# Autodesk Inventor assembly: TestRig
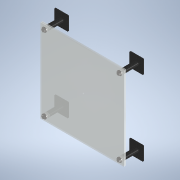
[picture p0: Inventor's stored thumbnail of the model, 180x180]
Saved by Autodesk Inventor 2020.3 (Build 243373010, 373A)
## iProperties
Created: 2020-10-30
Part Number: TestRig
Document SubType Name: Assembly
Designer: Naude Conradie
Author: Naude Conradie
## Documents named in this file (7)
- C:\Users\Naude Conradie\Desktop\Repository\Masters-Project\Models\Inventor\Testing Rig\TestRig.iam
- C:\Users\Naude Conradie\Desktop\Repository\Masters-Project\Models\Inventor\Testing Rig\Plate.ipt
- C:\Users\Naude Conradie\Desktop\Repository\Masters-Project\Models\Inventor\Testing Rig\PlateHoled.ipt
- C:\Users\Naude Conradie\Desktop\Repository\Masters-Project\Models\Inventor\Testing Rig\Leg.ipt
- C:\Users\Naude Conradie\Documents\Inventor\Content Center Files\R2020\en-US\ANSI B18.2.3.5M\ANSI B18.2.3.5M - M6 x 1 x 30.ipt
- C:\Users\Naude Conradie\Desktop\Repository\Masters-Project\Models\Inventor\Testing Rig\Washer.ipt
- C:\Users\Naude Conradie\Documents\Inventor\Content Center Files\R2020\en-US\IFI (3)\IFI - 6(9).ipt
## Components (22 placed, 6 different names)
1. Plate:1 — Mate:4, Flush:3, Mate:22, Mate:23, Mate:24, Mate:25, Mate:26, Mate:27, Mate:28, Mate:29, Mate:37, Mate:38, Mate:39, Mate:40, Mate:44, Mate:45, Mate:46, Mate:47, Angle:5, Angle:6, Angle:7, Angle:8
2. PlateHoled:1 — Mate:4, Flush:3, Mate:18, Mate:19, Mate:20, Mate:21, Angle:1, Angle:2, Angle:3, Angle:4, Mate:30, Mate:33, Mate:48, Mate:49, Mate:50
3. Leg:1 — Mate:18, Angle:1, Mate:35, Mate:43
4. Leg:2 — Mate:19, Angle:2, Mate:31, Mate:32
5. Leg:3 — Mate:20, Angle:3, Mate:34, Mate:42
6. Leg:4 — Mate:21, Angle:4, Mate:36, Mate:41
7. Hex Bolt - Metric M6 x 1 x 30:1 — Mate:51, Mate:57, Angle:7
8. Hex Bolt - Metric M6 x 1 x 30:2 — Mate:52, Mate:58, Angle:8
9. Hex Bolt - Metric M6 x 1 x 30:3 — Mate:53, Mate:55, Angle:5
10. Hex Bolt - Metric M6 x 1 x 30:4 — Mate:54, Mate:56, Angle:6
11. Washer:1 — Mate:22, Mate:27
12. Washer:2 — Mate:23, Mate:28
13. Washer:3 — Mate:25, Mate:29, Mate:30
14. Washer:4 — Mate:24, Mate:26
15. Round Test Washer (Metric) (IFI) 6:1 — Mate:31, Mate:32, Mate:33
16. Round Test Washer (Metric) (IFI) 6:2 — Mate:38, Mate:46, Mate:52, Mate:58
17. Round Test Washer (Metric) (IFI) 6:3 — Mate:39, Mate:45, Mate:51, Mate:57
18. Round Test Washer (Metric) (IFI) 6:4 — Mate:37, Mate:44, Mate:53, Mate:55
19. Round Test Washer (Metric) (IFI) 6:5 — Mate:40, Mate:47, Mate:54, Mate:56
20. Round Test Washer (Metric) (IFI) 6:6 — Mate:36, Mate:41, Mate:48
21. Round Test Washer (Metric) (IFI) 6:7 — Mate:35, Mate:43, Mate:50
22. Round Test Washer (Metric) (IFI) 6:8 — Mate:34, Mate:42, Mate:49
## Relationships (51: Mate 42, Angle 8, Flush 1)
- Mate:4: Plate:1 ↔ PlateHoled:1
- Flush:3: Plate:1 ↔ PlateHoled:1
- Mate:18: PlateHoled:1 ↔ Leg:1
- Mate:19: PlateHoled:1 ↔ Leg:2
- Mate:20: PlateHoled:1 ↔ Leg:3
- Mate:21: PlateHoled:1 ↔ Leg:4
- Angle:1 (0 deg): PlateHoled:1 ↔ Leg:1
- Angle:2 (0 deg): PlateHoled:1 ↔ Leg:2
- Angle:3 (0 deg): PlateHoled:1 ↔ Leg:3
- Angle:4 (0 deg): PlateHoled:1 ↔ Leg:4
- Mate:22: Plate:1 ↔ Washer:1
- Mate:23: Plate:1 ↔ Washer:2
- Mate:24: Plate:1 ↔ Washer:4
- Mate:25: Plate:1 ↔ Washer:3
- Mate:26: Plate:1 ↔ Washer:4
- Mate:27: Plate:1 ↔ Washer:1
- Mate:28: Plate:1 ↔ Washer:2
- Mate:29: Plate:1 ↔ Washer:3
- Mate:30: PlateHoled:1 ↔ Washer:3
- Mate:31: Leg:2 ↔ Round Test Washer (Metric) (IFI) 6:1
- Mate:32: Leg:2 ↔ Round Test Washer (Metric) (IFI) 6:1
- Mate:33: PlateHoled:1 ↔ Round Test Washer (Metric) (IFI) 6:1
- Mate:34: Leg:3 ↔ Round Test Washer (Metric) (IFI) 6:8
- Mate:35: Leg:1 ↔ Round Test Washer (Metric) (IFI) 6:7
- Mate:36: Leg:4 ↔ Round Test Washer (Metric) (IFI) 6:6
- Mate:37: Plate:1 ↔ Round Test Washer (Metric) (IFI) 6:4
- Mate:38: Plate:1 ↔ Round Test Washer (Metric) (IFI) 6:2
- Mate:39: Plate:1 ↔ Round Test Washer (Metric) (IFI) 6:3
- Mate:40: Plate:1 ↔ Round Test Washer (Metric) (IFI) 6:5
- Mate:41: Leg:4 ↔ Round Test Washer (Metric) (IFI) 6:6
- Mate:42: Leg:3 ↔ Round Test Washer (Metric) (IFI) 6:8
- Mate:43: Leg:1 ↔ Round Test Washer (Metric) (IFI) 6:7
- Mate:44: Plate:1 ↔ Round Test Washer (Metric) (IFI) 6:4
- Mate:45: Plate:1 ↔ Round Test Washer (Metric) (IFI) 6:3
- Mate:46: Plate:1 ↔ Round Test Washer (Metric) (IFI) 6:2
- Mate:47: Plate:1 ↔ Round Test Washer (Metric) (IFI) 6:5
- Mate:48: PlateHoled:1 ↔ Round Test Washer (Metric) (IFI) 6:6
- Mate:49: PlateHoled:1 ↔ Round Test Washer (Metric) (IFI) 6:8
- Mate:50: PlateHoled:1 ↔ Round Test Washer (Metric) (IFI) 6:7
- Mate:51: Hex Bolt - Metric M6 x 1 x 30:1 ↔ Round Test Washer (Metric) (IFI) 6:3
- Mate:52: Hex Bolt - Metric M6 x 1 x 30:2 ↔ Round Test Washer (Metric) (IFI) 6:2
- Mate:53: Hex Bolt - Metric M6 x 1 x 30:3 ↔ Round Test Washer (Metric) (IFI) 6:4
- Mate:54: Hex Bolt - Metric M6 x 1 x 30:4 ↔ Round Test Washer (Metric) (IFI) 6:5
- Mate:55: Hex Bolt - Metric M6 x 1 x 30:3 ↔ Round Test Washer (Metric) (IFI) 6:4
- Angle:5 (0 deg): Plate:1 ↔ Hex Bolt - Metric M6 x 1 x 30:3
- Mate:56: Hex Bolt - Metric M6 x 1 x 30:4 ↔ Round Test Washer (Metric) (IFI) 6:5
- Angle:6 (0 deg): Plate:1 ↔ Hex Bolt - Metric M6 x 1 x 30:4
- Mate:57: Hex Bolt - Metric M6 x 1 x 30:1 ↔ Round Test Washer (Metric) (IFI) 6:3
- Angle:7 (0 deg): Plate:1 ↔ Hex Bolt - Metric M6 x 1 x 30:1
- Mate:58: Hex Bolt - Metric M6 x 1 x 30:2 ↔ Round Test Washer (Metric) (IFI) 6:2
- Angle:8 (0 deg): Plate:1 ↔ Hex Bolt - Metric M6 x 1 x 30:2
